# Autodesk Inventor assembly: vange med trin
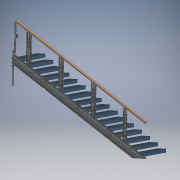
[picture p0: Inventor's stored thumbnail of the model, 180x180]
Saved by Autodesk Inventor 2018 (Build 220112000, 112)
## iProperties
Created: 2019-11-06
Part Number: vange med trin
Document SubType Name: Assembly
Designer: loppen
Author: loppen
## Documents named in this file (4)
- Z:\trappe\vange med trin.iam
- Z:\trappe\søjle+vange.iam
- Z:\trappe\trin\trin.iam
- Z:\trappe\trin\trin-top.iam
## Components (17 placed, 3 different names)
1. søjle+vange:1 [sub-assembly] — Mate:1, Mate:2, Mate:3, Mate:4, Mate:5, Mate:6, Mate:7, Mate:8, Mate:9, Mate:10, Mate:11, Mate:12, Mate:13, Mate:14, Mate:15, Mate:16, Mate:17, Mate:18, Mate:19, Mate:20, Mate:21, Mate:22, Mate:23, Mate:24, Mate:25, Mate:26, Mate:27, Mate:28, Mate:29, Mate:30, Mate:31, Mate:32, Mate:33, Mate:34, Mate:35, Mate:36, Mate:37, Mate:38, Mate:39, Mate:40, Mate:41, Mate:42, Mate:43, Mate:44, Mate:45, Mate:46, Mate:47, Mate:48, Mate:49
2. trin:1 [sub-assembly] — Mate:1, Mate:2, Mate:3
3. trin:2 [sub-assembly] — Mate:4, Mate:5, Mate:34
4. trin:3 [sub-assembly] — Mate:6, Mate:7, Mate:35
5. trin:4 [sub-assembly] — Mate:8, Mate:9, Mate:36
6. trin:5 [sub-assembly] — Mate:10, Mate:37, Mate:39
7. trin:6 [sub-assembly] — Mate:11, Mate:12, Mate:38
8. trin:7 [sub-assembly] — Mate:13, Mate:14, Mate:40
9. trin:8 [sub-assembly] — Mate:15, Mate:16, Mate:41, Mate:42
10. trin:9 [sub-assembly] — Mate:17, Mate:18, Mate:43
11. trin:10 [sub-assembly] — Mate:19, Mate:20, Mate:44
12. trin:11 [sub-assembly] — Mate:21, Mate:22, Mate:45
13. trin:12 [sub-assembly] — Mate:23, Mate:24, Mate:46
14. trin:13 [sub-assembly] — Mate:25, Mate:26, Mate:47
15. trin:14 [sub-assembly] — Mate:27, Mate:28, Mate:48
16. trin:15 [sub-assembly] — Mate:29, Mate:30, Mate:49
17. trin-top:1 [sub-assembly] — Mate:31, Mate:32, Mate:33
## Relationships (49: Mate 49)
- Mate:1: søjle+vange:1 ↔ trin:1
- Mate:2 (20 mm): søjle+vange:1 ↔ trin:1
- Mate:3: søjle+vange:1 ↔ trin:1
- Mate:4: søjle+vange:1 ↔ trin:2
- Mate:5: søjle+vange:1 ↔ trin:2
- Mate:6: søjle+vange:1 ↔ trin:3
- Mate:7: søjle+vange:1 ↔ trin:3
- Mate:8: søjle+vange:1 ↔ trin:4
- Mate:9: søjle+vange:1 ↔ trin:4
- Mate:10: søjle+vange:1 ↔ trin:5
- Mate:11: søjle+vange:1 ↔ trin:6
- Mate:12: søjle+vange:1 ↔ trin:6
- Mate:13: søjle+vange:1 ↔ trin:7
- Mate:14: søjle+vange:1 ↔ trin:7
- Mate:15: søjle+vange:1 ↔ trin:8
- Mate:16: søjle+vange:1 ↔ trin:8
- Mate:17: søjle+vange:1 ↔ trin:9
- Mate:18: søjle+vange:1 ↔ trin:9
- Mate:19: søjle+vange:1 ↔ trin:10
- Mate:20: søjle+vange:1 ↔ trin:10
- Mate:21: søjle+vange:1 ↔ trin:11
- Mate:22: søjle+vange:1 ↔ trin:11
- Mate:23: søjle+vange:1 ↔ trin:12
- Mate:24: søjle+vange:1 ↔ trin:12
- Mate:25: søjle+vange:1 ↔ trin:13
- Mate:26: søjle+vange:1 ↔ trin:13
- Mate:27: søjle+vange:1 ↔ trin:14
- Mate:28: søjle+vange:1 ↔ trin:14
- Mate:29: søjle+vange:1 ↔ trin:15
- Mate:30: søjle+vange:1 ↔ trin:15
- Mate:31: søjle+vange:1 ↔ trin-top:1
- Mate:32: søjle+vange:1 ↔ trin-top:1
- Mate:33 (20 mm): søjle+vange:1 ↔ trin-top:1
- Mate:34 (20 mm): søjle+vange:1 ↔ trin:2
- Mate:35 (20 mm): søjle+vange:1 ↔ trin:3
- Mate:36 (20 mm): søjle+vange:1 ↔ trin:4
- Mate:37 (20 mm): søjle+vange:1 ↔ trin:5
- Mate:38 (20 mm): søjle+vange:1 ↔ trin:6
- Mate:39: søjle+vange:1 ↔ trin:5
- Mate:40 (20 mm): søjle+vange:1 ↔ trin:7
- Mate:41 (20 mm): søjle+vange:1 ↔ trin:8
- Mate:42 (20 mm): søjle+vange:1 ↔ trin:8
- Mate:43 (20 mm): søjle+vange:1 ↔ trin:9
- Mate:44 (20 mm): søjle+vange:1 ↔ trin:10
- Mate:45 (20 mm): søjle+vange:1 ↔ trin:11
- Mate:46 (20 mm): søjle+vange:1 ↔ trin:12
- Mate:47 (20 mm): søjle+vange:1 ↔ trin:13
- Mate:48 (20 mm): søjle+vange:1 ↔ trin:14
- Mate:49 (20 mm): søjle+vange:1 ↔ trin:15
